# Autodesk Inventor assembly: FO_020_318_4F_2_03
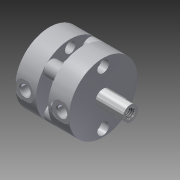
[picture p0: Inventor's stored thumbnail of the model, 180x180]
Saved by Autodesk Inventor 2013 (Build 170138000, 138)
## iProperties
Created: 2013-06-25
Part Number: FO_020_318_4F_2_03
Document SubType Name: Assembly
Designer: mvarma
Author: mvarma
## Documents named in this file (10)
- C:\Users\mvarma\Desktop\GRT 2013-2014 Gearbox\Mark 4\Pneumatic\FO_020_318_4F_2_03.iam
- C:\Users\mvarma\Desktop\GRT 2013-2014 Gearbox\Mark 4\Pneumatic\Pneumatic Parts\1.ipt
- C:\Users\mvarma\Desktop\GRT 2013-2014 Gearbox\Mark 4\Pneumatic\Pneumatic Parts\2.ipt
- C:\Users\mvarma\Desktop\GRT 2013-2014 Gearbox\Mark 4\Pneumatic\Pneumatic Parts\3.ipt
- C:\Users\mvarma\Desktop\GRT 2013-2014 Gearbox\Mark 4\Pneumatic\Pneumatic Parts\4.ipt
- C:\Users\mvarma\Desktop\GRT 2013-2014 Gearbox\Mark 4\Pneumatic\Pneumatic Parts\5.ipt
- C:\Users\mvarma\Desktop\GRT 2013-2014 Gearbox\Mark 4\Pneumatic\Pneumatic Parts\6.ipt
- C:\Users\mvarma\Desktop\GRT 2013-2014 Gearbox\Mark 4\Pneumatic\Pneumatic Parts\7.ipt
- C:\Users\mvarma\Desktop\GRT 2013-2014 Gearbox\Mark 4\Pneumatic\Pneumatic Parts\8.ipt
- C:\Users\mvarma\Desktop\GRT 2013-2014 Gearbox\Mark 4\Pneumatic\Pneumatic Parts\9.ipt
## Components (9 placed, 9 different names)
1. 1:1 — Mate:1, Mate:2, Mate:3, Mate:4, Mate:5, Mate:6, Mate:7, Mate:8, Mate:13, Mate:14
2. 2:1 — Mate:12, Mate:13, Mate:14, Flush:2
3. 3:1 — Mate:9, Mate:10, Mate:15
4. 4:1 — Mate:11, Flush:1
5. 5:1 — Mate:11, Flush:1, Mate:12, Flush:2
6. 6:1 — Mate:5, Mate:6, Mate:15
7. 7:1 — Mate:7, Mate:8, Mate:10
8. 8:1 — Mate:3, Mate:4, Mate:9
9. 9:1 — Mate:1, Mate:2
## Relationships (17: Mate 15, Flush 2)
- Mate:1: 1:1 ↔ 9:1
- Mate:2: 1:1 ↔ 9:1
- Mate:3: 1:1 ↔ 8:1
- Mate:4: 1:1 ↔ 8:1
- Mate:5: 1:1 ↔ 6:1
- Mate:6: 1:1 ↔ 6:1
- Mate:7: 1:1 ↔ 7:1
- Mate:8: 1:1 ↔ 7:1
- Mate:9: 3:1 ↔ 8:1
- Mate:10: 3:1 ↔ 7:1
- Mate:11: 4:1 ↔ 5:1
- Flush:1: 4:1 ↔ 5:1
- Mate:12: 2:1 ↔ 5:1
- Mate:13: 1:1 ↔ 2:1
- Mate:14: 1:1 ↔ 2:1
- Flush:2: 2:1 ↔ 5:1
- Mate:15: 3:1 ↔ 6:1
